# Autodesk Inventor assembly: TouchAssembly
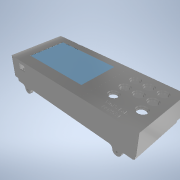
[picture p0: Inventor's stored thumbnail of the model, 180x180]
Saved by Autodesk Inventor 2020 (Build 240168000, 168)
## iProperties
Created: 2021-05-02
Part Number: TouchAssembly
Document SubType Name: Assembly
Designer: 10300812
Author: 10300812
## Documents named in this file (4)
- C:\Users\10300812\Documents\GitHub\Philips-PM2534\TouchAssembly.iam
- C:\Users\10300812\Documents\GitHub\Philips-PM2534\FrontCoverTouch.ipt
- C:\Users\10300812\Documents\GitHub\Philips-PM2534\MB1191.ipt
- C:\Users\10300812\Documents\GitHub\Philips-PM2534\DisplayCover.ipt
## Components (3 placed, 3 different names)
1. FrontCoverTouch:1 — Mate:2, Mate:3, Mate:4, Mate:5, Mate:6, Flush:1
2. MB1191:1 — Mate:2, Mate:3, Mate:4
3. DisplayCover:1 — Mate:5, Mate:6, Flush:1
## Relationships (6: Mate 5, Flush 1)
- Mate:2: FrontCoverTouch:1 ↔ MB1191:1
- Mate:3: FrontCoverTouch:1 ↔ MB1191:1
- Mate:4: FrontCoverTouch:1 ↔ MB1191:1
- Mate:5: FrontCoverTouch:1 ↔ DisplayCover:1
- Mate:6: FrontCoverTouch:1 ↔ DisplayCover:1
- Flush:1: FrontCoverTouch:1 ↔ DisplayCover:1
